# Autodesk Inventor assembly: Dodecahedron
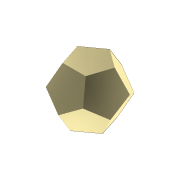
[picture p0: Inventor's stored thumbnail of the model, 180x180]
Saved by Autodesk Inventor 2022.2 (Build 262287010, 287A)
## iProperties
Created: 2022-12-30
Part Number: Dodecahedron
Document SubType Name: Assembly
Designer: User
Author: User
## Documents named in this file (2)
- C:\Users\User\Desktop\InventorTutorial prof Stancesu\Part20Dodecahedron\Dodecahedron.iam
- C:\Users\User\Desktop\InventorTutorial prof Stancesu\Part20Dodecahedron\Face.ipt
## Components (12 placed, 1 different names)
1. Face:1 — Mate:1, Mate:2, Mate:3, Mate:6, Mate:7, Mate:13
2. Face:2 — Mate:1, Mate:2, Mate:4, Mate:16, Mate:17, Mate:19
3. Face:3 — Mate:13, Mate:16, Mate:18
4. Face:4 — Mate:15, Mate:17, Mate:21, Mate:22
5. Face:5 — Mate:14, Mate:18
6. Face:6 — Mate:11, Mate:12, Mate:20
7. Face:7 — Mate:3, Mate:4, Mate:5, Mate:12, Mate:15
8. Face:8 — Mate:5, Mate:6, Mate:8, Mate:10, Mate:11
9. Face:9 — Mate:7, Mate:8, Mate:9, Mate:14
10. Face:10 — Mate:9, Mate:10
11. Face:11 — Mate:20, Mate:22
12. Face:12 — Mate:19, Mate:21
## Relationships (22: Mate 22)
- Mate:1: Face:1 ↔ Face:2
- Mate:2: Face:1 ↔ Face:2
- Mate:3: Face:1 ↔ Face:7
- Mate:4: Face:2 ↔ Face:7
- Mate:5: Face:7 ↔ Face:8
- Mate:6: Face:1 ↔ Face:8
- Mate:7: Face:1 ↔ Face:9
- Mate:8: Face:8 ↔ Face:9
- Mate:9: Face:9 ↔ Face:10
- Mate:10: Face:8 ↔ Face:10
- Mate:11: Face:6 ↔ Face:8
- Mate:12: Face:6 ↔ Face:7
- Mate:13: Face:1 ↔ Face:3
- Mate:14: Face:5 ↔ Face:9
- Mate:15: Face:4 ↔ Face:7
- Mate:16: Face:2 ↔ Face:3
- Mate:17: Face:2 ↔ Face:4
- Mate:18: Face:3 ↔ Face:5
- Mate:19: Face:2 ↔ Face:12
- Mate:20: Face:6 ↔ Face:11
- Mate:21: Face:4 ↔ Face:12
- Mate:22: Face:4 ↔ Face:11
